# Autodesk Inventor assembly: X_Führung
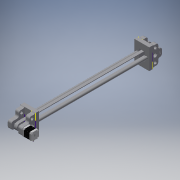
[picture p0: Inventor's stored thumbnail of the model, 180x180]
Saved by Autodesk Inventor 2019 (Build 230136000, 136)
## iProperties
Created: 2018-08-19
Part Number: X_Führung
Document SubType Name: Assembly
Designer: Julia
Author: Julia
## Documents named in this file (6)
- C:\Users\Julia\Documents\Inventor\3d_Drucker_v02\X_Führung.iam
- C:\Users\Julia\Documents\Inventor\3d_Drucker_v02\Y_Slider_mit_Schrittmotor.iam
- C:\Users\Julia\Documents\Inventor\3d_Drucker_v02\Y_Slider.iam
- C:\Users\Julia\Documents\Inventor\3d_Drucker_v02\X_Führungsstange.ipt
- C:\Users\Julia\Documents\Inventor\3d_Drucker_v02\X_Zahnriemen.ipt
- C:\Users\Julia\Documents\Inventor\3d_Drucker_v02\Schrittmotor_Nema_17.ipt
## Components (6 placed, 5 different names)
1. Y_Slider_mit_Schrittmotor:1 [sub-assembly] — Mate:5, Mate:6, Mate:7, Mate:11, Mate:12, Mate:13, Angle:3
2. Y_Slider:1 [sub-assembly] — Mate:1, Mate:2, Mate:3, Mate:4, Angle:1, Angle:2, Flush:1
3. X_Führungsstange:1 — Mate:2, Mate:3, Mate:5
4. X_Zahnriemen:1 — Angle:1, Angle:2, Flush:1, Mate:11
5. X_Führungsstange:2 — Mate:1, Mate:4, Mate:6, Mate:7
6. Schrittmotor_Nema_17:1 — Mate:12, Mate:13, Angle:3
## Relationships (14: Mate 10, Angle 3, Flush 1)
- Mate:1: Y_Slider:1 ↔ X_Führungsstange:2
- Mate:2: Y_Slider:1 ↔ X_Führungsstange:1
- Mate:3: Y_Slider:1 ↔ X_Führungsstange:1
- Mate:4: Y_Slider:1 ↔ X_Führungsstange:2
- Mate:5: Y_Slider_mit_Schrittmotor:1 ↔ X_Führungsstange:1
- Mate:6: Y_Slider_mit_Schrittmotor:1 ↔ X_Führungsstange:2
- Mate:7: Y_Slider_mit_Schrittmotor:1 ↔ X_Führungsstange:2
- Angle:1 (0 deg): Y_Slider:1 ↔ X_Zahnriemen:1
- Angle:2 (0 deg): Y_Slider:1 ↔ X_Zahnriemen:1
- Flush:1: Y_Slider:1 ↔ X_Zahnriemen:1
- Mate:11: Y_Slider_mit_Schrittmotor:1 ↔ X_Zahnriemen:1
- Mate:12: Y_Slider_mit_Schrittmotor:1 ↔ Schrittmotor_Nema_17:1
- Mate:13: Y_Slider_mit_Schrittmotor:1 ↔ Schrittmotor_Nema_17:1
- Angle:3 (0 deg): Y_Slider_mit_Schrittmotor:1 ↔ Schrittmotor_Nema_17:1
